# Autodesk Inventor assembly: Frame
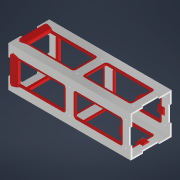
[picture p0: Inventor's stored thumbnail of the model, 180x180]
Saved by Autodesk Inventor 2022 (Build 260153000, 153)
## iProperties
Created: 2022-07-14
Part Number: Frame
Document SubType Name: Assembly
Designer: ForseFire
Author: ForseFire
## Documents named in this file (4)
- C:\Users\ForseFire\Desktop\Frame.iam
- C:\Users\ForseFire\Desktop\InventorFull\Frame.ipt
- C:\Users\ForseFire\Desktop\InventorFull\SolarpanelAdapter.ipt
- C:\Users\ForseFire\Desktop\InventorFull\SolarpanelAdapter_bot.ipt
## Components (9 placed, 3 different names)
1. Frame:1 — Mate:1, Mate:2, Mate:3, Mate:4, Mate:5, Mate:6, Mate:7, Mate:8, Mate:9, Mate:10, Mate:11, Mate:12, Mate:13, Mate:14, Mate:15, Mate:16, Mate:17, Mate:18, Mate:19, Mate:20, Mate:21, Mate:22
2. SolarpanelAdapter:1 — Mate:18, Mate:19
3. SolarpanelAdapter_bot:1 — Mate:20, Mate:21, Mate:22
4. SolarpanelAdapter:2 — Mate:12, Mate:13, Mate:14
5. SolarpanelAdapter_bot:2 — Mate:15, Mate:16, Mate:17
6. SolarpanelAdapter:3 — Mate:7, Mate:8, Mate:9
7. SolarpanelAdapter_bot:3 — Mate:10, Mate:11
8. SolarpanelAdapter:4 — Mate:1, Mate:2, Mate:3
9. SolarpanelAdapter_bot:4 — Mate:4, Mate:5, Mate:6
## Relationships (22: Mate 22)
- Mate:1: Frame:1 ↔ SolarpanelAdapter:4
- Mate:2: Frame:1 ↔ SolarpanelAdapter:4
- Mate:3: Frame:1 ↔ SolarpanelAdapter:4
- Mate:4: Frame:1 ↔ SolarpanelAdapter_bot:4
- Mate:5: Frame:1 ↔ SolarpanelAdapter_bot:4
- Mate:6: Frame:1 ↔ SolarpanelAdapter_bot:4
- Mate:7: Frame:1 ↔ SolarpanelAdapter:3
- Mate:8: Frame:1 ↔ SolarpanelAdapter:3
- Mate:9: Frame:1 ↔ SolarpanelAdapter:3
- Mate:10: Frame:1 ↔ SolarpanelAdapter_bot:3
- Mate:11: Frame:1 ↔ SolarpanelAdapter_bot:3
- Mate:12: Frame:1 ↔ SolarpanelAdapter:2
- Mate:13: Frame:1 ↔ SolarpanelAdapter:2
- Mate:14: Frame:1 ↔ SolarpanelAdapter:2
- Mate:15: Frame:1 ↔ SolarpanelAdapter_bot:2
- Mate:16: Frame:1 ↔ SolarpanelAdapter_bot:2
- Mate:17: Frame:1 ↔ SolarpanelAdapter_bot:2
- Mate:18: Frame:1 ↔ SolarpanelAdapter:1
- Mate:19: Frame:1 ↔ SolarpanelAdapter:1
- Mate:20: Frame:1 ↔ SolarpanelAdapter_bot:1
- Mate:21: Frame:1 ↔ SolarpanelAdapter_bot:1
- Mate:22: Frame:1 ↔ SolarpanelAdapter_bot:1
